# Autodesk Inventor assembly: C-SHFMQ20
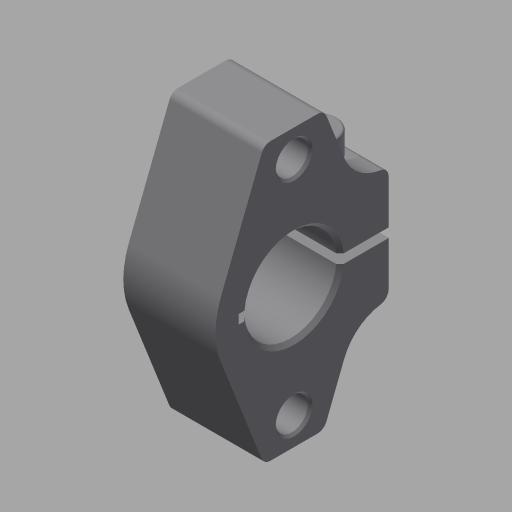
[picture p0: Inventor's stored thumbnail of the model, 512x512]
Saved by Autodesk Inventor 2024 (Build 280153000, 153)
## iProperties
Category: PARTsolutions
Company: MISUMI
Created: 2023-06-23
Part Number: C-SHFMQ20
Catalog Web Link: www.cadenas.de
Description: C-SHFMQ-Economy Shaft Supports - Flanged Slit (Precision Cast) Standard Type
Vendor: MISUMI
Document SubType Name: Assembly
Designer: psAdmin
Manufacturer: MISUMI
Mass: 23.8706 g
Surface Area: 90.211 cm^2
Volume: 23.8706 cm^3
Density: 1 g/cm^3
PSOL_IDENT_0: {$CADENAS_DATA/23d-libs/misumi/metric/02_shaft_supports/c_shfmq_asmtab.prj},173 {VTYP=3D},{STYP=ASST
PSOL_IDENT_1: AB},{NB=C-SHFMQ20},{LINA=C-SHFMQ20},{NN=C-SHFMQ},{DATE=12.09.2022 01:30:54},{GEOMDATE=16.03.2021 06:
PSOL_IDENT_2: 16:19},{VERSION=},{LINEID=40},{WBVAR=},{WBNUMERIC=}  {NB=C-SHFMQ20},{LINA=C-SHFMQ20},{KT=DUMMY},{PN=
PSOL_IDENT_3: C-SHFMQ20},{D=20},{L=60},{T=20},{L1=48},{H=37.5},{DD=7.0},{M1=M5},{M=5},{H1=13},{DH=5.5},{R1=17.0},{
PSOL_IDENT_4: R2=10},{R3=2},{L2=25.0},{L3=12.0},{B=2.0},{LH=15.0},{RH=5},{LM=20},{C=0.5},{PPATH=c_shfmq/c_shfmq_as
PSOL_IDENT_5: mtpl.prj}
NB: C-SHFMQ20
NN: C-SHFMQ
NT: Economy Shaft Supports - Flanged Slit (Precision Cast) Standard Type
NBSYN: $PN.
LINA: C-SHFMQ20
CATALOG: Misumi
PN: C-SHFMQ20
D: 20
L: 60
T: 20
L1: 48
H: 37.5
DD: 7
M1: M5
SUPPLIER: MISUMI
ARTICLENO: C-SHFMQ20
BOMINFO: C-SHFMQ20
CREATOR: CADENAS GmbH
Title: C-SHFMQ20
Author: Cadenas PARTsolutions
Comments: Economy Shaft Supports - Flanged Slit (Precision Cast) Standard Type
## Documents named in this file (3)
- C:\Users\zegi\OneDrive - Kyushu University\KURT\2023キャチロボ\cad\000_parts_zegi\parts\shaft_holder\C-SHFMQ20\AIS2022\C-SHFMQ20.iam
- C:\Users\zegi\OneDrive - Kyushu University\KURT\2023キャチロボ\cad\000_parts_zegi\parts\shaft_holder\C-SHFMQ20\AIS2022\C-SHFMQ20_b.ipt
- C:\Users\zegi\OneDrive - Kyushu University\KURT\2023キャチロボ\cad\000_parts_zegi\parts\shaft_holder\C-SHFMQ20\AIS2022\Slotted head cap screw ISO 4762 - M5x20.ipt
## Components (2 placed, 2 different names)
1. C-SHFMQ20_b:1 — to_bolt_Z@1 <-> IP1_Z@2
2. Slotted head cap screw ISO 4762 - M5x20:1 — to_bolt_Z@1 <-> IP1_Z@2
## Relationships (1: Mate 1)
- to_bolt_Z@1 <-> IP1_Z@2 [Mate]: C-SHFMQ20_b:1 ↔ Slotted head cap screw ISO 4762 - M5x20:1
